# Autodesk Inventor assembly: lifterCI
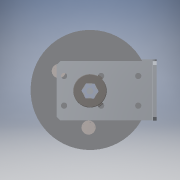
[picture p0: Inventor's stored thumbnail of the model, 180x180]
Saved by Autodesk Inventor 2017 (Build 210142000, 142)
## iProperties
Created: 2017-03-08
Part Number: lifterCI
Document SubType Name: Assembly
Designer: kingb
Author: kingb
## Documents named in this file (8)
- C:\Users\kingb\Desktop\CAD\lifterCI.iam
- C:\Users\kingb\Desktop\CAD\spoolEnd.ipt
- C:\Users\kingb\Desktop\CAD\spoolChurro.ipt
- C:\Users\kingb\Desktop\CAD\FHTS 0.25-20-0.75_FHTS 0.25-20-G-0.75-C.ipt
- C:\Users\kingb\Desktop\CAD\Churro 20250.ipt
- C:\Users\kingb\Desktop\CAD\FR8ZZ Hex Bearing.ipt
- C:\Users\kingb\Desktop\CAD\am-2954 AM14U2 2x3 Hole Bracket.ipt
- C:\Users\kingb\Desktop\CAD\7552K500_HEXAGONAL-BORE CLAMP-ON SHAFT COLLAR.ipt
## Components (18 placed, 7 different names)
1. spoolChurro:1 — Insert:1, Insert:4, Angle:2, Angle:6, Angle:9
2. spoolEnd:1 — Insert:1, Insert:2, Insert:3, Insert:7, Insert:8, Insert:9, Mate:1, Mate:2, Mate:18
3. spoolChurro:2 — Insert:3, Insert:6, Angle:3, Angle:5, Angle:7
4. spoolChurro:3 — Insert:2, Insert:5, Angle:1, Angle:4, Angle:8
5. spoolEnd:2 — Insert:4, Insert:5, Insert:6, Angle:1, Angle:2, Angle:3, Insert:10, Insert:11, Insert:12, Tangent:1, Mate:17
6. FHTS 0.25-20-0.75_FHTS 0.25-20-G-0.75-C:1 — Insert:12, Angle:4
7. FHTS 0.25-20-0.75_FHTS 0.25-20-G-0.75-C:2 — Insert:10, Angle:6
8. FHTS 0.25-20-0.75_FHTS 0.25-20-G-0.75-C:3 — Insert:11, Angle:5
9. FHTS 0.25-20-0.75_FHTS 0.25-20-G-0.75-C:4 — Insert:7, Angle:9
10. FHTS 0.25-20-0.75_FHTS 0.25-20-G-0.75-C:5 — Insert:9, Angle:8
11. FHTS 0.25-20-0.75_FHTS 0.25-20-G-0.75-C:6 — Insert:8, Angle:7
12. Churro 20250:1 — Mate:1, Mate:2, Mate:3, Mate:4, Mate:5, Mate:6, Mate:13, Mate:14, Mate:15, Mate:16
13. FR8ZZ Hex Bearing:1 — Mate:3, Mate:4, Mate:10, Tangent:2, Mate:12
14. FR8ZZ Hex Bearing:2 — Mate:5, Mate:6, Mate:9, Tangent:3, Mate:11
15. am-2954 AM14U2 2x3 Hole Bracket:1 — Mate:7, Mate:10, Tangent:2
16. am-2954 AM14U2 2x3 Hole Bracket:2 — Mate:8, Mate:9, Tangent:3
17. 7552K500_HEXAGONAL-BORE CLAMP-ON SHAFT COLLAR:1 — Mate:12, Mate:13, Mate:14, Mate:17
18. 7552K500_HEXAGONAL-BORE CLAMP-ON SHAFT COLLAR:2 — Mate:11, Mate:15, Mate:16, Mate:18
## Relationships (44: Mate 18, Insert 12, Angle 10, Tangent 3, Flush 1)
- Insert:1: spoolChurro:1 ↔ spoolEnd:1
- Insert:2: spoolEnd:1 ↔ spoolChurro:3
- Insert:3: spoolEnd:1 ↔ spoolChurro:2
- Insert:4: spoolChurro:1 ↔ spoolEnd:2
- Insert:5: spoolChurro:3 ↔ spoolEnd:2
- Insert:6: spoolChurro:2 ↔ spoolEnd:2
- Angle:1 (0 deg): spoolChurro:3 ↔ spoolEnd:2
- Angle:2 (0 deg): spoolChurro:1 ↔ spoolEnd:2
- Angle:3 (0 deg): spoolChurro:2 ↔ spoolEnd:2
- Insert:7: spoolEnd:1 ↔ FHTS 0.25-20-0.75_FHTS 0.25-20-G-0.75-C:4
- Insert:8: spoolEnd:1 ↔ FHTS 0.25-20-0.75_FHTS 0.25-20-G-0.75-C:6
- Insert:9: spoolEnd:1 ↔ FHTS 0.25-20-0.75_FHTS 0.25-20-G-0.75-C:5
- Insert:10: spoolEnd:2 ↔ FHTS 0.25-20-0.75_FHTS 0.25-20-G-0.75-C:2
- Insert:11: spoolEnd:2 ↔ FHTS 0.25-20-0.75_FHTS 0.25-20-G-0.75-C:3
- Insert:12: spoolEnd:2 ↔ FHTS 0.25-20-0.75_FHTS 0.25-20-G-0.75-C:1
- Angle:4 (0 deg): spoolChurro:3 ↔ FHTS 0.25-20-0.75_FHTS 0.25-20-G-0.75-C:1
- Angle:5 (0 deg): spoolChurro:2 ↔ FHTS 0.25-20-0.75_FHTS 0.25-20-G-0.75-C:3
- Angle:6 (0 deg): spoolChurro:1 ↔ FHTS 0.25-20-0.75_FHTS 0.25-20-G-0.75-C:2
- Angle:7 (0 deg): spoolChurro:2 ↔ FHTS 0.25-20-0.75_FHTS 0.25-20-G-0.75-C:6
- Angle:8 (0 deg): spoolChurro:3 ↔ FHTS 0.25-20-0.75_FHTS 0.25-20-G-0.75-C:5
- Angle:9 (0 deg): spoolChurro:1 ↔ FHTS 0.25-20-0.75_FHTS 0.25-20-G-0.75-C:4
- Mate:1: spoolEnd:1 ↔ Churro 20250:1
- Mate:2: spoolEnd:1 ↔ Churro 20250:1
- Angle:10 (0 deg)
- Tangent:1: spoolEnd:2
- Flush:1 (-6.35 mm)
- Mate:3: Churro 20250:1 ↔ FR8ZZ Hex Bearing:1
- Mate:4: Churro 20250:1 ↔ FR8ZZ Hex Bearing:1
- Mate:5: Churro 20250:1 ↔ FR8ZZ Hex Bearing:2
- Mate:6: Churro 20250:1 ↔ FR8ZZ Hex Bearing:2
- Mate:7: am-2954 AM14U2 2x3 Hole Bracket:1
- Mate:8: am-2954 AM14U2 2x3 Hole Bracket:2
- Mate:9: FR8ZZ Hex Bearing:2 ↔ am-2954 AM14U2 2x3 Hole Bracket:2
- Mate:10: FR8ZZ Hex Bearing:1 ↔ am-2954 AM14U2 2x3 Hole Bracket:1
- Tangent:2 (11.1125 mm): FR8ZZ Hex Bearing:1 ↔ am-2954 AM14U2 2x3 Hole Bracket:1
- Tangent:3 (11.1125 mm): FR8ZZ Hex Bearing:2 ↔ am-2954 AM14U2 2x3 Hole Bracket:2
- Mate:11: FR8ZZ Hex Bearing:2 ↔ 7552K500_HEXAGONAL-BORE CLAMP-ON SHAFT COLLAR:2
- Mate:12: FR8ZZ Hex Bearing:1 ↔ 7552K500_HEXAGONAL-BORE CLAMP-ON SHAFT COLLAR:1
- Mate:13: Churro 20250:1 ↔ 7552K500_HEXAGONAL-BORE CLAMP-ON SHAFT COLLAR:1
- Mate:14: Churro 20250:1 ↔ 7552K500_HEXAGONAL-BORE CLAMP-ON SHAFT COLLAR:1
- Mate:15: Churro 20250:1 ↔ 7552K500_HEXAGONAL-BORE CLAMP-ON SHAFT COLLAR:2
- Mate:16: Churro 20250:1 ↔ 7552K500_HEXAGONAL-BORE CLAMP-ON SHAFT COLLAR:2
- Mate:17: spoolEnd:2 ↔ 7552K500_HEXAGONAL-BORE CLAMP-ON SHAFT COLLAR:1
- Mate:18: spoolEnd:1 ↔ 7552K500_HEXAGONAL-BORE CLAMP-ON SHAFT COLLAR:2
